# Autodesk Inventor assembly: moldspace
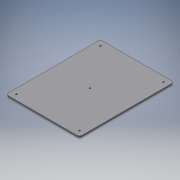
[picture p0: Inventor's stored thumbnail of the model, 180x180]
Saved by Autodesk Inventor 2017 (Build 210142000, 142)
## iProperties
Part Number: moldspace
Material: 一般
Document SubType Name: Assembly
Designer: highs
Author: highs
## Documents named in this file (3)
- C:\Users\highs\Desktop\学校\中の島\moldspace.iam
- C:\Users\highs\Desktop\学校\卒業研究\コバンザメユニット\UVGmold2.ipt
- C:\Users\highs\Desktop\学校\卒業研究\コバンザメユニット\UVGmold3.ipt
## Components (2 placed, 2 different names)
1. UVGmold2:1 — メイト:1, メイト:2, メイト:3
2. UVGmold3:1 — メイト:1, メイト:2, メイト:3
## Relationships (3: Mate 3)
- メイト:1 [Mate]: UVGmold2:1 ↔ UVGmold3:1
- メイト:2 [Mate]: UVGmold2:1 ↔ UVGmold3:1
- メイト:3 [Mate]: UVGmold2:1 ↔ UVGmold3:1
